# Autodesk Inventor assembly: TabletMountAssembly
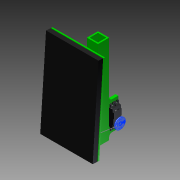
[picture p0: Inventor's stored thumbnail of the model, 180x180]
Saved by Autodesk Inventor 2012 (Build 160160000, 160)
## iProperties
Created: 2013-07-16
Part Number: TabletMountAssembly
Document SubType Name: Assembly
Designer: joe_000
Author: joe_000
## Documents named in this file (7)
- C:\dev\telepresenceRobot\mechanical\TabletMountAssembly.iam
- C:\dev\telepresenceRobot\mechanical\TableMount-Base.ipt
- C:\dev\telepresenceRobot\mechanical\Servo.ipt
- C:\dev\telepresenceRobot\mechanical\Servo-Horn.ipt
- C:\dev\telepresenceRobot\mechanical\Nexus7.ipt
- C:\dev\telepresenceRobot\mechanical\TableMount-Holder.ipt
- C:\dev\telepresenceRobot\mechanical\TableMount-ServoWire.ipt
## Components (6 placed, 6 different names)
1. TableMount-Base:1 — Mate:1, Insert:2, Insert:3, Insert:4
2. Servo:1 — Insert:1, Mate:1, Insert:2, Insert:3
3. Servo-Horn:1 — Insert:1, Insert:5
4. Nexus7:1 — Mate:2
5. TableMount-Holder:1 — Insert:4, Mate:2, Tangent:1
6. TableMount-ServoWire:1 — Insert:5, Tangent:1
## Relationships (8: Insert 5, Mate 2, Tangent 1)
- Insert:1: Servo:1 ↔ Servo-Horn:1
- Mate:1: TableMount-Base:1 ↔ Servo:1
- Insert:2: TableMount-Base:1 ↔ Servo:1
- Insert:3: TableMount-Base:1 ↔ Servo:1
- Insert:4: TableMount-Base:1 ↔ TableMount-Holder:1
- Mate:2: Nexus7:1 ↔ TableMount-Holder:1
- Insert:5: Servo-Horn:1 ↔ TableMount-ServoWire:1
- Tangent:1: TableMount-Holder:1 ↔ TableMount-ServoWire:1
